# Autodesk Inventor assembly: ABD_Version_0.1_leftleg
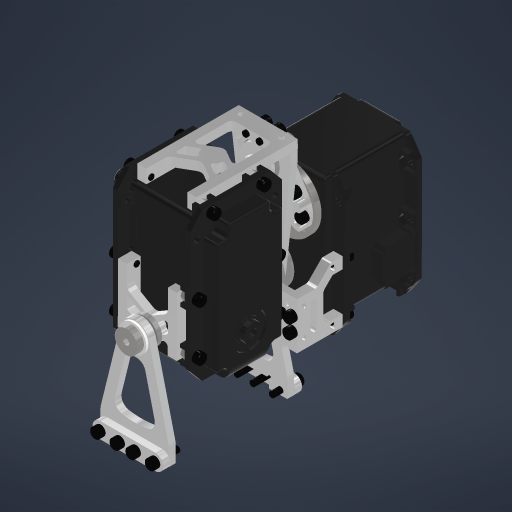
[picture p0: Inventor's stored thumbnail of the model, 512x512]
Saved by Autodesk Inventor 2024.3 (Build 283343000, 343)
## iProperties
Created: 2024-01-23
Part Number: ABD_Version_0.1_leftleg
Document SubType Name: Assembly
Designer: ASUS
Mass: 357.136 g
Surface Area: 604.848 cm^2
Volume: 181.423 cm^3
Density: 1.96853 g/cm^3
Author: ASUS
## Documents named in this file (6)
- C:\Users\ASUS\Desktop\test\v2_Frame\ABD_V2_Left_OP.iam
- C:\Users\ASUS\Desktop\test\v2_Frame\Roll_Fixation_Set.iam
- C:\Users\ASUS\Desktop\test\v2_Frame\ABD_MX_64_Roll_Fixation_Set.iam
- C:\Users\ASUS\Desktop\test\v2_Frame\ABD_MX_64_Slider_Fixation_Set_Right2Horn.iam
- C:\Users\ASUS\Desktop\test\v2_Frame\Crank_Slider_Fixer.iam
- C:\Users\ASUS\Desktop\test\v2_Frame\ABD_Slider_Set_v2.iam
## Components (5 placed, 5 different names)
1. Roll_Fixation_Set:1 [sub-assembly] — 삽입:5, 각도:1, 메이트:54
2. ABD_MX_64_Roll_Fixation_Set:1 [sub-assembly] — 메이트:2, 메이트:3, 삽입:5, 각도:1
3. ABD_MX_64_Slider_Fixation_Set_Right2Horn:1 [sub-assembly] — 메이트:2, 메이트:3, 메이트:52, 메이트:53
4. Crank_Slider_Fixer:6 [sub-assembly] — 메이트:52, 메이트:53, 삽입:7
5. ABD_Slider_Set_v2:1 [sub-assembly] — 삽입:7, 메이트:54
## Relationships (8: Mate 5, Insert 2, Angle 1)
- 메이트:2 [Mate] (0.05 mm): ABD_MX_64_Roll_Fixation_Set:1 ↔ ABD_MX_64_Slider_Fixation_Set_Right2Horn:1
- 메이트:3 [Mate]: ABD_MX_64_Roll_Fixation_Set:1 ↔ ABD_MX_64_Slider_Fixation_Set_Right2Horn:1
- 삽입:5 [Insert]: Roll_Fixation_Set:1 ↔ ABD_MX_64_Roll_Fixation_Set:1
- 각도:1 [Angle] (0 deg): Roll_Fixation_Set:1 ↔ ABD_MX_64_Roll_Fixation_Set:1
- 메이트:52 [Mate]: ABD_MX_64_Slider_Fixation_Set_Right2Horn:1 ↔ Crank_Slider_Fixer:6
- 메이트:53 [Mate]: ABD_MX_64_Slider_Fixation_Set_Right2Horn:1 ↔ Crank_Slider_Fixer:6
- 삽입:7 [Insert]: Crank_Slider_Fixer:6 ↔ ABD_Slider_Set_v2:1
- 메이트:54 [Mate]: Roll_Fixation_Set:1 ↔ ABD_Slider_Set_v2:1
